# Autodesk Inventor assembly: CAR_012_CarouselDriveAssembly
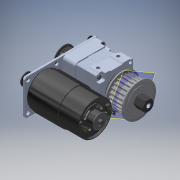
[picture p0: Inventor's stored thumbnail of the model, 180x180]
Saved by Autodesk Inventor 2018 (Build 220112000, 112)
## iProperties
Created: 2020-02-01
Part Number: CAR_012_CarouselDriveAssembly
Document SubType Name: Assembly
Designer: user
Author: user
## Documents named in this file (4)
- C:\Users\user\Documents\GrabCAD\New folder\Build season\CAR_012_CarouselDriveAssembly.iam
- C:\Users\user\Documents\GrabCAD\New folder\Build season\CAR_011_VersaPlanetary_v2_Single_Stage_10_1_with_775_Series_Reverse.iam
- C:\Users\user\Documents\GrabCAD\New folder\Build season\CHA_007_DrivenPulleyAssembly.iam
- C:\Users\user\Documents\GrabCAD\New folder\Build season\CAR_013_24t_x_15mm_Wide_Aluminum_Pulley_HTD_5mm_1_2_Hex_217-4101.ipt
## Components (3 placed, 3 different names)
1. CAR_011_VersaPlanetary_v2_Single_Stage_10_1_with_775_Series_Reverse:1 [sub-assembly] — Mate:1, Mate:2, Flush:1, Angle:1, Tangent:1, Mate:3, Mate:4, Angle:2, Tangent:2, Mate:5
2. CHA_007_DrivenPulleyAssembly:1 [sub-assembly] — Mate:1, Mate:2, Flush:1
3. CAR_013_24t_x_15mm_Wide_Aluminum_Pulley_HTD_5mm_1_2_Hex_217-4101:1 — Mate:3, Mate:4, Mate:5
## Relationships (10: Mate 5, Angle 2, Tangent 2, Flush 1)
- Mate:1: CAR_011_VersaPlanetary_v2_Single_Stage_10_1_with_775_Series_Reverse:1 ↔ CHA_007_DrivenPulleyAssembly:1
- Mate:2: CAR_011_VersaPlanetary_v2_Single_Stage_10_1_with_775_Series_Reverse:1 ↔ CHA_007_DrivenPulleyAssembly:1
- Flush:1: CAR_011_VersaPlanetary_v2_Single_Stage_10_1_with_775_Series_Reverse:1 ↔ CHA_007_DrivenPulleyAssembly:1
- Angle:1 (0 deg): CAR_011_VersaPlanetary_v2_Single_Stage_10_1_with_775_Series_Reverse:1
- Tangent:1: CAR_011_VersaPlanetary_v2_Single_Stage_10_1_with_775_Series_Reverse:1
- Mate:3: CAR_011_VersaPlanetary_v2_Single_Stage_10_1_with_775_Series_Reverse:1 ↔ CAR_013_24t_x_15mm_Wide_Aluminum_Pulley_HTD_5mm_1_2_Hex_217-4101:1
- Mate:4: CAR_011_VersaPlanetary_v2_Single_Stage_10_1_with_775_Series_Reverse:1 ↔ CAR_013_24t_x_15mm_Wide_Aluminum_Pulley_HTD_5mm_1_2_Hex_217-4101:1
- Angle:2 (0 deg): CAR_011_VersaPlanetary_v2_Single_Stage_10_1_with_775_Series_Reverse:1
- Tangent:2: CAR_011_VersaPlanetary_v2_Single_Stage_10_1_with_775_Series_Reverse:1
- Mate:5 (6.35 mm): CAR_011_VersaPlanetary_v2_Single_Stage_10_1_with_775_Series_Reverse:1 ↔ CAR_013_24t_x_15mm_Wide_Aluminum_Pulley_HTD_5mm_1_2_Hex_217-4101:1
